# Autodesk Inventor assembly: motor-mount
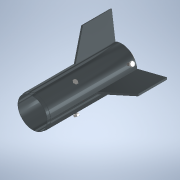
[picture p0: Inventor's stored thumbnail of the model, 180x180]
Saved by Autodesk Inventor 2021 (Build 250183000, 183)
## iProperties
Created: 2021-03-30
Part Number: motor-mount
Document SubType Name: Assembly
Designer: samlo
Author: samlo
## Documents named in this file (7)
- C:\Users\samlo\Documents\airframev1\Design\motor-mount.iam
- C:\Users\samlo\Documents\airframev1\Design\tail.ipt
- C:\Users\samlo\Documents\airframev1\Design\motor-mount-top.ipt
- C:\Users\samlo\Documents\airframev1\Design\motor-standin.ipt
- C:\Users\samlo\Documents\airframev1\Design\motor-mount-bottom.ipt
- C:\Users\samlo\OneDrive\Documents\Inventor\Content Center Files\R2021\en-US\IFI 502(18)\IFI 502 - M4x0.7 x 13(2) D.ipt
- C:\Users\samlo\OneDrive\Documents\Inventor\Content Center Files\R2021\en-US\IFI 502(18)\IFI 502 - M4x0.7 x 20(2) D.ipt
## Components (10 placed, 6 different names)
1. tail:1 — Mate:1, Mate:2, Mate:5, Mate:6, Mate:7, Mate:8, Mate:9, Mate:12
2. motor-mount-top:1 — Mate:1, Mate:2, Mate:3, Mate:4, Mate:10, Mate:11
3. motor-standin:1 — Mate:3, Mate:4
4. motor-mount-bottom:1 — Mate:5, Mate:6
5. Fully Upset Hex Head Tapping Screw - Type D - Metric M4x0.7 x 13:1 — Mate:8
6. Fully Upset Hex Head Tapping Screw - Type D - Metric M4x0.7 x 13:2 — Mate:9
7. Fully Upset Hex Head Tapping Screw - Type D - Metric M4x0.7 x 13:3 — Mate:7
8. Fully Upset Hex Head Tapping Screw - Type D - Metric M4x0.7 x 20:4 — Mate:12
9. Fully Upset Hex Head Tapping Screw - Type D - Metric M4x0.7 x 20:5 — Mate:11
10. Fully Upset Hex Head Tapping Screw - Type D - Metric M4x0.7 x 20:6 — Mate:10
## Relationships (12: Mate 12)
- Mate:1: tail:1 ↔ motor-mount-top:1
- Mate:2: tail:1 ↔ motor-mount-top:1
- Mate:3: motor-mount-top:1 ↔ motor-standin:1
- Mate:4: motor-mount-top:1 ↔ motor-standin:1
- Mate:5: tail:1 ↔ motor-mount-bottom:1
- Mate:6: tail:1 ↔ motor-mount-bottom:1
- Mate:7: tail:1 ↔ Fully Upset Hex Head Tapping Screw - Type D - Metric M4x0.7 x 13:3
- Mate:8: tail:1 ↔ Fully Upset Hex Head Tapping Screw - Type D - Metric M4x0.7 x 13:1
- Mate:9: tail:1 ↔ Fully Upset Hex Head Tapping Screw - Type D - Metric M4x0.7 x 13:2
- Mate:10: motor-mount-top:1 ↔ Fully Upset Hex Head Tapping Screw - Type D - Metric M4x0.7 x 20:6
- Mate:11: motor-mount-top:1 ↔ Fully Upset Hex Head Tapping Screw - Type D - Metric M4x0.7 x 20:5
- Mate:12: tail:1 ↔ Fully Upset Hex Head Tapping Screw - Type D - Metric M4x0.7 x 20:4
